# Autodesk Inventor assembly: Board Fail
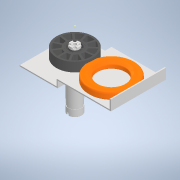
[picture p0: Inventor's stored thumbnail of the model, 180x180]
Saved by Autodesk Inventor 2020.3 (Build 243373010, 373A)
## iProperties
Created: 2020-09-26
Part Number: Board Fail
Document SubType Name: Assembly
Designer: Owner
Author: Owner
## Documents named in this file (8)
- C:\Users\Owner\Documents\Board Fail.iam
- C:\Users\Owner\Documents\Single Sided board.ipt
- C:\Users\Owner\Downloads\1206-0016-0004 assembly\1206-0016-0004 assembly.ipt
- C:\Users\Owner\Downloads\am-3563 4IN 8mm Round Compliant Wheel REV2.ipt
- C:\Users\Owner\Downloads\5202-0002-0003\5202-0002-0003 part.ipt
- C:\Users\Owner\Downloads\545636 assembly\545636 assembly.ipt
- C:\Users\Owner\Downloads\545456_1\545456.ipt
- C:\Users\Owner\Downloads\am-4300 Ring.ipt
## Components (8 placed, 7 different names)
1. 1206-0016-0004 assembly:1 — Mate:1, Mate:2, Mate:3, Mate:4, Mate:9, Mate:11
2. am-3563 4IN 8mm Round Compliant Wheel REV2:1 — Mate:7, Mate:8
3. Single Sided board:1 — Mate:1, Mate:2, Mate:3, Mate:5, Mate:13, Tangent:1
4. 5202-0002-0003 part:1 — Mate:4, Mate:5
5. 545636 assembly:1 — Mate:9, Mate:11, Mate:12
6. 545456:1 — Mate:7
7. 545456:2 — Mate:8, Mate:12
8. am-4300 Ring:1 — Mate:13, Tangent:1
## Relationships (12: Mate 11, Tangent 1)
- Mate:1: 1206-0016-0004 assembly:1 ↔ Single Sided board:1
- Mate:2: 1206-0016-0004 assembly:1 ↔ Single Sided board:1
- Mate:3: 1206-0016-0004 assembly:1 ↔ Single Sided board:1
- Mate:4: 1206-0016-0004 assembly:1 ↔ 5202-0002-0003 part:1
- Mate:5: Single Sided board:1 ↔ 5202-0002-0003 part:1
- Mate:7: am-3563 4IN 8mm Round Compliant Wheel REV2:1 ↔ 545456:1
- Mate:8: am-3563 4IN 8mm Round Compliant Wheel REV2:1 ↔ 545456:2
- Mate:9: 1206-0016-0004 assembly:1 ↔ 545636 assembly:1
- Mate:11: 1206-0016-0004 assembly:1 ↔ 545636 assembly:1
- Mate:12: 545636 assembly:1 ↔ 545456:2
- Mate:13: Single Sided board:1 ↔ am-4300 Ring:1
- Tangent:1: Single Sided board:1 ↔ am-4300 Ring:1
